# Autodesk Inventor assembly: Proto2
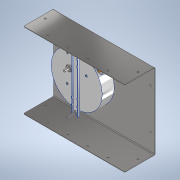
[picture p0: Inventor's stored thumbnail of the model, 180x180]
Saved by Autodesk Inventor 2020 (Build 240168000, 168)
## iProperties
Created: 2020-06-17
Part Number: Proto2
Document SubType Name: Assembly
Designer: Juan
Author: Juan
## Documents named in this file (10)
- C:\Users\Juan\Desktop\CNAF\Plato Grueso\Proto2.iam
- C:\Users\Juan\Desktop\CNAF\Caja Base CNAF\3D STEP\Ensamblaje_v5.iam
- C:\Users\Juan\Desktop\CNAF\Plato Grueso\Sello Plato Oring2155.ipt
- C:\Users\Juan\Desktop\CNAF\Plato Grueso\Platogrueso.ipt
- C:\Users\Juan\Desktop\CNAF\Plato Grueso\Termocupla.ipt
- C:\Users\Juan\Desktop\CNAF\Plato Grueso\Calefactor630W.ipt
- C:\Users\Juan\Desktop\CNAF\Plato Grueso\Prisionero DIN913-M5x5.ipt
- C:\Users\Juan\Desktop\CNAF\Plato Grueso\Parker DIN912-M3x45.ipt
- C:\Users\Juan\Desktop\CNAF\Plato Grueso\Barra fijación calefactor.ipt
- C:\Users\Juan\Desktop\CNAF\Plato Grueso\Tuerca DIN934-M3.ipt
## Components (12 placed, 9 different names)
1. Ensamblaje_v5:1 [sub-assembly] — Cylindrical:1, Cylindrical:5, Planar:1, Angle:1
2. Sello Plato Oring2155:1 — Cylindrical:1, Cylindrical:2
3. Platogrueso:1 — Cylindrical:2, Cylindrical:3, Rotational:1, Mate:1, Cylindrical:4, Mate:2
4. Termocupla:1 — Cylindrical:3
5. Calefactor630W:1 — Mate:1
6. Prisionero DIN913-M5x5:1 — Cylindrical:4
7. Prisionero DIN913-M5x5:2 — Rotational:1
8. Parker DIN912-M3x45:1 — Cylindrical:5, Cylindrical:6
9. Parker DIN912-M3x45:2 — Planar:1
10. Barra fijación calefactor:1 — Mate:2, Cylindrical:6, Angle:1, Insert:1, Insert:2
11. Tuerca DIN934-M3:1 — Insert:1
12. Tuerca DIN934-M3:2 — Insert:2
## Relationships (13: CylindricalJoint 6, Mate 2, Insert 2, RevoluteJoint 1, PlanarJoint 1, Angle 1)
- Cylindrical:1: Ensamblaje_v5:1 ↔ Sello Plato Oring2155:1
- Cylindrical:2: Sello Plato Oring2155:1 ↔ Platogrueso:1
- Cylindrical:3: Platogrueso:1 ↔ Termocupla:1
- Rotational:1 [RevoluteJoint]: Platogrueso:1 ↔ Prisionero DIN913-M5x5:2
- Mate:1: Platogrueso:1 ↔ Calefactor630W:1
- Cylindrical:4: Platogrueso:1 ↔ Prisionero DIN913-M5x5:1
- Cylindrical:5: Ensamblaje_v5:1 ↔ Parker DIN912-M3x45:1
- Planar:1: Ensamblaje_v5:1 ↔ Parker DIN912-M3x45:2
- Mate:2: Platogrueso:1 ↔ Barra fijación calefactor:1
- Cylindrical:6: Parker DIN912-M3x45:1 ↔ Barra fijación calefactor:1
- Angle:1 (0 deg): Ensamblaje_v5:1 ↔ Barra fijación calefactor:1
- Insert:1: Barra fijación calefactor:1 ↔ Tuerca DIN934-M3:1
- Insert:2: Barra fijación calefactor:1 ↔ Tuerca DIN934-M3:2
